# Autodesk Inventor assembly: Backpack
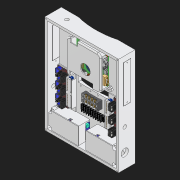
[picture p0: Inventor's stored thumbnail of the model, 180x180]
Saved by Autodesk Inventor 2017 SP1 (Build 210196100, 196)
## iProperties
Created: 2017-09-05
Part Number: Backpack
Document SubType Name: Assembly
Designer: Zach
Author: Zach
## Documents named in this file (15)
- C:\Users\Zach\Documents\GitHub\tr1\src\Body\Chest Assembly\Backpack Assembly\Backpack.iam
- C:\Users\Zach\Documents\GitHub\tr1\src\Body\Chest Assembly\Backpack Assembly\BP001b.ipt
- C:\Users\Zach\Documents\GitHub\tr1\src\Body\Chest Assembly\Backpack Assembly\BP002b.ipt
- C:\Users\Zach\Documents\GitHub\tr1\src\Body\Chest Assembly\Backpack Assembly\BP003.ipt
- C:\Users\Zach\Documents\GitHub\tr1\src\Body\Chest Assembly\Backpack Assembly\BP004.ipt
- C:\Users\Zach\Documents\GitHub\tr1\src\Body\Chest Assembly\Backpack Assembly\BP005.ipt
- C:\Users\Zach\Documents\GitHub\tr1\src\Body\Chest Assembly\Backpack Assembly\BP006.ipt
- C:\Users\Zach\Documents\GitHub\tr1\lib\Terminal Block 4\Клемная колодка ТВ-2504L 600V-25A\Клемная колодка ТВ-2504L 600V-25A.iam
- C:\Users\Zach\Documents\GitHub\tr1\lib\Arduino Nano\Arduino Nano V3 assemble.iam
- C:\Users\Zach\Documents\GitHub\tr1\lib\NVIDIA Jetson TK1\Jetson_TK1_FabD_3D.iam
- C:\Users\Zach\Documents\GitHub\tr1\lib\Arduino Mega 2560\Arduino Mega 2560.ipt
- C:\Users\Zach\Documents\GitHub\tr1\src\Body\Chest Assembly\Backpack Assembly\BP007.ipt
- C:\Users\Zach\Documents\GitHub\tr1\lib\L298n H Bridge\L298N\07j5423_1546306-8.ipt
- C:\Users\Zach\Documents\GitHub\tr1\lib\L298n Driver\l298n.ipt
- C:\Users\Zach\Documents\GitHub\tr1\src\Body\Chest Assembly\Backpack Assembly\BP008.ipt
## Components (27 placed, 14 different names)
1. BP001b:1 — Mate:1, Mate:2, Mate:3, Mate:6, Mate:8, Mate:9, Mate:11, Mate:13, Mate:15, Mate:19, Mate:20, Mate:21, Mate:22, Mate:23, Flush:1, Mate:24, Mate:25, Mate:26, Mate:35, Mate:36, Mate:37, Mate:38, Mate:39, Mate:42, Mate:43, Mate:44, Mate:45, Mate:46, Mate:56, Mate:57, Mate:58, Mate:78, Mate:79, Mate:80, Mate:81, Mate:82
2. BP002b:1 — Mate:1, Mate:2, Mate:3
3. BP003:1 — Mate:15, Mate:36, Mate:37, Mate:50, Mate:51, Mate:52, Mate:53, Mate:54, Mate:55, Mate:65, Angle:2, Mate:66, Mate:67, Mate:68, Mate:69, Mate:70
4. BP004:1 — Mate:6, Mate:44, Mate:45
5. BP005:1 — Mate:8, Mate:9, Mate:20
6. BP006:1 — Mate:11, Mate:13, Mate:21
7. BP003:2 — Mate:19, Mate:27, Mate:28, Mate:29, Mate:30, Mate:31, Mate:32, Mate:38, Mate:39, Mate:59, Mate:60, Angle:1, Mate:61, Mate:62, Mate:63, Mate:64
8. Клемная колодка ТВ-2504L 600V-25A:1 [sub-assembly] — Mate:24, Mate:25, Mate:26
9. Arduino Nano V3 assemble:1 [sub-assembly] — Mate:27, Mate:28, Mate:29
10. Arduino Nano V3 assemble:2 [sub-assembly] — Mate:30, Mate:31, Mate:32
11. Jetson_TK1_FabD_3D:1 [sub-assembly] — Mate:35, Mate:42, Mate:43
12. Arduino Mega 2560:1 — Mate:49, Mate:75, Mate:76, Mate:77
13. Arduino Mega 2560:2 — Mate:83, Mate:84, Mate:85, Mate:86
14. BP007:1 — Mate:46, Mate:49, Mate:72, Mate:73, Mate:74, Mate:75, Mate:76, Mate:77, Mate:78, Mate:79, Mate:87, Mate:88, Mate:89
15. Arduino Nano V3 assemble:3 [sub-assembly] — Mate:53, Mate:54, Mate:55
16. Arduino Nano V3 assemble:4 [sub-assembly] — Mate:50, Mate:51, Mate:52
17. 07j5423_1546306-8:1 — Mate:56, Mate:57, Mate:58
18. l298n:1 — Mate:59, Mate:60, Angle:1, Flush:3
19. l298n:2 — Mate:62, Mate:63, Flush:2, Flush:3
20. l298n:3 — Mate:61, Mate:64, Flush:2
21. l298n:4 — Mate:67, Mate:70, Flush:4, Flush:5
22. l298n:5 — Mate:68, Mate:69, Flush:5
23. l298n:6 — Mate:65, Angle:2, Mate:66, Flush:4
24. BP008:1 — Mate:72, Mate:73, Mate:74
25. BP007:2 — Mate:80, Mate:81, Mate:82, Mate:83, Mate:84, Mate:85, Mate:86, Mate:90, Mate:91, Mate:92
26. BP008:2 — Mate:87, Mate:88, Mate:89
27. BP008:3 — Mate:90, Mate:91, Mate:92
## Relationships (83: Mate 76, Flush 5, Angle 2)
- Mate:1: BP001b:1 ↔ BP002b:1
- Mate:2: BP001b:1 ↔ BP002b:1
- Mate:3: BP001b:1 ↔ BP002b:1
- Mate:6: BP001b:1 ↔ BP004:1
- Mate:8: BP001b:1 ↔ BP005:1
- Mate:9: BP001b:1 ↔ BP005:1
- Mate:11: BP001b:1 ↔ BP006:1
- Mate:13: BP001b:1 ↔ BP006:1
- Mate:15: BP001b:1 ↔ BP003:1
- Mate:19: BP001b:1 ↔ BP003:2
- Mate:20: BP001b:1 ↔ BP005:1
- Mate:21: BP001b:1 ↔ BP006:1
- Mate:22: BP001b:1
- Mate:23: BP001b:1
- Flush:1 (200 mm): BP001b:1
- Mate:24: BP001b:1 ↔ Клемная колодка ТВ-2504L 600V-25A:1
- Mate:25: BP001b:1 ↔ Клемная колодка ТВ-2504L 600V-25A:1
- Mate:26: BP001b:1 ↔ Клемная колодка ТВ-2504L 600V-25A:1
- Mate:27: BP003:2 ↔ Arduino Nano V3 assemble:1
- Mate:28: BP003:2 ↔ Arduino Nano V3 assemble:1
- Mate:29 (0.6 mm): BP003:2 ↔ Arduino Nano V3 assemble:1
- Mate:30: BP003:2 ↔ Arduino Nano V3 assemble:2
- Mate:31: BP003:2 ↔ Arduino Nano V3 assemble:2
- Mate:32 (0.6 mm): BP003:2 ↔ Arduino Nano V3 assemble:2
- Mate:35: BP001b:1 ↔ Jetson_TK1_FabD_3D:1
- Mate:36: BP001b:1 ↔ BP003:1
- Mate:37: BP001b:1 ↔ BP003:1
- Mate:38: BP001b:1 ↔ BP003:2
- Mate:39: BP001b:1 ↔ BP003:2
- Mate:42: BP001b:1 ↔ Jetson_TK1_FabD_3D:1
- Mate:43: BP001b:1 ↔ Jetson_TK1_FabD_3D:1
- Mate:44: BP001b:1 ↔ BP004:1
- Mate:45: BP001b:1 ↔ BP004:1
- Mate:46: BP001b:1 ↔ BP007:1
- Mate:49: Arduino Mega 2560:1 ↔ BP007:1
- Mate:50: BP003:1 ↔ Arduino Nano V3 assemble:4
- Mate:51 (0.6 mm): BP003:1 ↔ Arduino Nano V3 assemble:4
- Mate:52: BP003:1 ↔ Arduino Nano V3 assemble:4
- Mate:53: BP003:1 ↔ Arduino Nano V3 assemble:3
- Mate:54 (0.6 mm): BP003:1 ↔ Arduino Nano V3 assemble:3
- Mate:55: BP003:1 ↔ Arduino Nano V3 assemble:3
- Mate:56: BP001b:1 ↔ 07j5423_1546306-8:1
- Mate:57: BP001b:1 ↔ 07j5423_1546306-8:1
- Mate:58: BP001b:1 ↔ 07j5423_1546306-8:1
- Mate:59: BP003:2 ↔ l298n:1
- Mate:60: BP003:2 ↔ l298n:1
- Angle:1 (180 deg): BP003:2 ↔ l298n:1
- Mate:61: BP003:2 ↔ l298n:3
- Mate:62: BP003:2 ↔ l298n:2
- Mate:63: BP003:2 ↔ l298n:2
- Mate:64: BP003:2 ↔ l298n:3
- Flush:2: l298n:2 ↔ l298n:3
- Flush:3: l298n:1 ↔ l298n:2
- Mate:65: BP003:1 ↔ l298n:6
- Angle:2 (180 deg): BP003:1 ↔ l298n:6
- Mate:66: BP003:1 ↔ l298n:6
- Mate:67: BP003:1 ↔ l298n:4
- Mate:68: BP003:1 ↔ l298n:5
- Mate:69: BP003:1 ↔ l298n:5
- Mate:70: BP003:1 ↔ l298n:4
- Flush:4: l298n:4 ↔ l298n:6
- Flush:5: l298n:4 ↔ l298n:5
- Mate:72: BP007:1 ↔ BP008:1
- Mate:73: BP007:1 ↔ BP008:1
- Mate:74: BP007:1 ↔ BP008:1
- Mate:75: Arduino Mega 2560:1 ↔ BP007:1
- Mate:76: Arduino Mega 2560:1 ↔ BP007:1
- Mate:77: Arduino Mega 2560:1 ↔ BP007:1
- Mate:78: BP001b:1 ↔ BP007:1
- Mate:79: BP001b:1 ↔ BP007:1
- Mate:80: BP001b:1 ↔ BP007:2
- Mate:81: BP001b:1 ↔ BP007:2
- Mate:82: BP001b:1 ↔ BP007:2
- Mate:83: Arduino Mega 2560:2 ↔ BP007:2
- Mate:84: Arduino Mega 2560:2 ↔ BP007:2
- Mate:85: Arduino Mega 2560:2 ↔ BP007:2
- Mate:86: Arduino Mega 2560:2 ↔ BP007:2
- Mate:87: BP007:1 ↔ BP008:2
- Mate:88: BP007:1 ↔ BP008:2
- Mate:89: BP007:1 ↔ BP008:2
- Mate:90: BP007:2 ↔ BP008:3
- Mate:91: BP007:2 ↔ BP008:3
- Mate:92: BP007:2 ↔ BP008:3
